# Autodesk Inventor assembly: Unit_SR-W
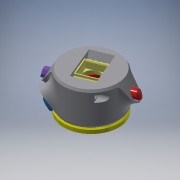
[picture p0: Inventor's stored thumbnail of the model, 180x180]
Saved by Autodesk Inventor 2018 (Build 220112000, 112)
## iProperties
Created: 2018-04-24
Part Number: Unit_SR-W
Material: 一般
Document SubType Name: Assembly
Designer: sktom
Author: sktom
## Documents named in this file (9)
- D:\cloudstrage\OneDrive\CADMech\HbSizeSMech\UnitWrist\Unit_SR-W.iam
- D:\cloudstrage\OneDrive\CADMech\HbSizeSMech\UnitWrist\Parts_SR-W\SR-W-04.ipt
- D:\cloudstrage\OneDrive\CADMech\HbSizeSMech\UnitWrist\Parts_SR-W\SR-W-05.ipt
- D:\cloudstrage\OneDrive\CADMech\HbSizeSMech\UnitWrist\Parts_SR-W\SR-W-02.ipt
- D:\cloudstrage\OneDrive\CADMech\HbSizeSMech\UnitWrist\Parts_SR-W\SR-W-08.ipt
- D:\cloudstrage\OneDrive\CADMech\HbSizeSMech\UnitWrist\Parts_SR-W\SR-W-01.ipt
- D:\cloudstrage\OneDrive\CADMech\HbSizeSMech\UnitWrist\Parts_SR-W\SR-W-03.ipt
- D:\cloudstrage\OneDrive\CADMech\HbSizeSMech\UnitWrist\Parts_SR-W\SR-W-06.ipt
- D:\cloudstrage\OneDrive\CADMech\HbSizeSMech\UnitWrist\Parts_SR-W\SR-W-07.ipt
## Components (8 placed, 8 different names)
1. SR-W-01:1 — リジッド:1
2. SR-W-02:1 — 挿入:3, 挿入:4, 挿入:5, リジッド:1, 円柱状:1, 挿入:6, 円柱状:2, メイト:1
3. SR-W-03:1 — 円柱状:1, 挿入:6
4. SR-W-04:1 — 挿入:1, 挿入:2, 挿入:3
5. SR-W-05:1 — 挿入:1, 挿入:2
6. SR-W-06:1 — リジッド:2
7. SR-W-07:1 — リジッド:2, 円柱状:2, メイト:1
8. SR-W-08:1 — 挿入:4, 挿入:5
## Relationships (11: Insert 6, WeldJoint 2, CylindricalJoint 2, Mate 1)
- 挿入:1 [Insert]: SR-W-04:1 ↔ SR-W-05:1
- 挿入:2 [Insert]: SR-W-04:1 ↔ SR-W-05:1
- 挿入:3 [Insert]: SR-W-02:1 ↔ SR-W-04:1
- 挿入:4 [Insert]: SR-W-02:1 ↔ SR-W-08:1
- 挿入:5 [Insert]: SR-W-02:1 ↔ SR-W-08:1
- リジッド:1 [WeldJoint]: SR-W-01:1 ↔ SR-W-02:1
- 円柱状:1 [CylindricalJoint]: SR-W-02:1 ↔ SR-W-03:1
- 挿入:6 [Insert]: SR-W-02:1 ↔ SR-W-03:1
- リジッド:2 [WeldJoint]: SR-W-06:1 ↔ SR-W-07:1
- 円柱状:2 [CylindricalJoint]: SR-W-02:1 ↔ SR-W-07:1
- メイト:1 [Mate] (0.5 mm): SR-W-02:1 ↔ SR-W-07:1
